# Autodesk Inventor assembly: tiltservomount_std
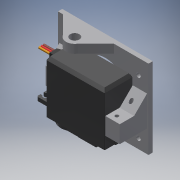
[picture p0: Inventor's stored thumbnail of the model, 180x180]
Saved by Autodesk Inventor 2017 (Build 210142000, 142)
## iProperties
Created: 2017-03-10
Part Number: tiltservomount_std
Description: FreeCAD Model
Document SubType Name: Assembly
Designer: Naga
Authority: Unknown
Sending System: FreeCAD
Preprocessor: Open CASCADE STEP processor 6.8
Title: E:/GDrive/IEEE CS/SoutheastCon2017/Cad/tilt/step/tiltservomount_std.step
Author: Author
## Documents named in this file (3)
- E:\GDrive\IEEE CS\SoutheastCon2017\Cad\tilt\step\tiltservomount_std.iam
- E:\GDrive\IEEE CS\SoutheastCon2017\Cad\tilt\step\difference004.ipt
- E:\GDrive\IEEE CS\SoutheastCon2017\Cad\Motors\MG995_Servo.iam
## Components (2 placed, 2 different names)
1. 3 — Mate:1, Mate:2, Flush:1
2. MG995_Servo:1 [sub-assembly] — Mate:1, Mate:2, Flush:1
## Relationships (3: Mate 2, Flush 1)
- Mate:1: 3 ↔ MG995_Servo:1
- Mate:2: 3 ↔ MG995_Servo:1
- Flush:1: 3 ↔ MG995_Servo:1
